# Autodesk Inventor assembly: pingmodule-y
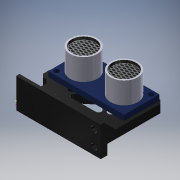
[picture p0: Inventor's stored thumbnail of the model, 180x180]
Saved by Autodesk Inventor 2018.3 (Build 223284000, 284)
## iProperties
Created: 2018-11-27
Part Number: pingmodule-y
Material: 一般
Document SubType Name: Assembly
Designer: shun2
Author: shun2
## Documents named in this file (3)
- C:\Users\shun2\OneDrive\おそらく最新版(2018.7.31)\pingmodule-y.iam
- C:\Users\shun2\OneDrive\おそらく最新版(2018.7.31)\ping.ipt
- C:\Users\shun2\OneDrive\おそらく最新版(2018.7.31)\PingCover-y.ipt
## Components (2 placed, 2 different names)
1. ping:1 — メイト:1, メイト:2, メイト:3
2. PingCover-y:1 — メイト:1, メイト:2, メイト:3
## Relationships (3: Mate 3)
- メイト:1 [Mate] (0.5 mm): ping:1 ↔ PingCover-y:1
- メイト:2 [Mate]: ping:1 ↔ PingCover-y:1
- メイト:3 [Mate]: ping:1 ↔ PingCover-y:1
